# Autodesk Inventor assembly: end-support-assembly
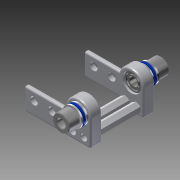
[picture p0: Inventor's stored thumbnail of the model, 180x180]
Saved by Autodesk Inventor 2015 (Build 190159000, 159)
## iProperties
Created: 2013-07-07
Part Number: end-support-assembly
Document SubType Name: Assembly
Designer: mhgreen
Author: mhgreen
## Documents named in this file (7)
- C:\Users\Michael\Dropbox\autocad\openbuild\end-support-assembly.iam
- C:\Users\Michael\Dropbox\autocad\openbuild\parts\13mmBearingBracketLeft.ipt
- C:\Users\Michael\Dropbox\autocad\openbuild\parts\13mmBearingBracketRight.ipt
- C:\Users\Michael\Dropbox\autocad\openbuild\parts\STEP\Imported Components\Bearing_6x13x5_a_7y_5mpss1306\Bearing_6x13x5_a_7y_5mpss1306.ipt
- C:\Users\Michael\Dropbox\autocad\openbuild\parts\STEP\Imported Components\6mmThrust_a_7z_7m0614st\6mmThrust_a_7z_7m0614st.ipt
- C:\Users\Michael\Dropbox\autocad\openbuild\parts\STEP\Imported Components\6mmShaftCollar_a_7c_2m112060\6mmShaftCollar_a_7c_2m112060.ipt
- C:\Users\Michael\Dropbox\autocad\openbuild\parts\STEP\Imported Components\M4_30MM_95947A062\M4_30MM_95947A062.ipt
## Components (10 placed, 6 different names)
1. 13mmBearingBracketLeft:1 — Insert:1, Mate:7
2. 13mmBearingBracketRight:1 — Insert:2, Insert:6, Insert:8, Insert:9
3. Bearing_6x13x5_a_7y_5mpss1306:1 — Insert:2
4. Bearing_6x13x5_a_7y_5mpss1306:2 — Insert:1
5. 6mmThrust_a_7z_7m0614st:1 — Insert:6, Insert:7
6. 6mmThrust_a_7z_7m0614st:2 — Mate:7, Insert:5
7. 6mmShaftCollar_a_7c_2m112060:1 — Insert:5
8. 6mmShaftCollar_a_7c_2m112060:2 — Insert:7
9. M4_30MM_95947A062:1 — Insert:8
10. M4_30MM_95947A062:2 — Insert:9
## Relationships (8: Insert 7, Mate 1)
- Insert:1: 13mmBearingBracketLeft:1 ↔ Bearing_6x13x5_a_7y_5mpss1306:2
- Insert:2: 13mmBearingBracketRight:1 ↔ Bearing_6x13x5_a_7y_5mpss1306:1
- Mate:7: 13mmBearingBracketLeft:1 ↔ 6mmThrust_a_7z_7m0614st:2
- Insert:5: 6mmThrust_a_7z_7m0614st:2 ↔ 6mmShaftCollar_a_7c_2m112060:1
- Insert:6: 13mmBearingBracketRight:1 ↔ 6mmThrust_a_7z_7m0614st:1
- Insert:7: 6mmThrust_a_7z_7m0614st:1 ↔ 6mmShaftCollar_a_7c_2m112060:2
- Insert:8: 13mmBearingBracketRight:1 ↔ M4_30MM_95947A062:1
- Insert:9: 13mmBearingBracketRight:1 ↔ M4_30MM_95947A062:2
